# Autodesk Inventor assembly: HoderCutter
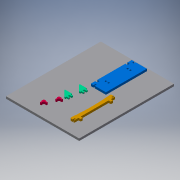
[picture p0: Inventor's stored thumbnail of the model, 180x180]
Saved by Autodesk Inventor 2019 (Build 230136000, 136)
## iProperties
Created: 2018-12-05
Part Number: HoderCutter
Document SubType Name: Assembly
Designer: Administrator
Author: Administrator
## Documents named in this file (6)
- H:\Space\Monster Holder\HoderCutter.iam
- H:\Space\Monster Holder\CuttingBoardPrint.ipt
- H:\Space\Monster Holder\MonsterHolderBase.ipt
- H:\Space\Monster Holder\MonsterHolderSupport1.ipt
- H:\Space\Monster Holder\MonsterHolderSupport2.ipt
- H:\Space\Monster Holder\MonsterHolderSupport3.ipt
## Components (7 placed, 5 different names)
1. CuttingBoardPrint:1 — Mate:1, Mate:2, Mate:3, Mate:4, Mate:5, Mate:6
2. MonsterHolderBase:1 — Mate:1
3. MonsterHolderSupport1:1 — Mate:6
4. MonsterHolderSupport1:2 — Mate:5
5. MonsterHolderSupport2:1 — Mate:2
6. MonsterHolderSupport3:1 — Mate:4
7. MonsterHolderSupport3:2 — Mate:3
## Relationships (6: Mate 6)
- Mate:1: CuttingBoardPrint:1 ↔ MonsterHolderBase:1
- Mate:2: CuttingBoardPrint:1 ↔ MonsterHolderSupport2:1
- Mate:3: CuttingBoardPrint:1 ↔ MonsterHolderSupport3:2
- Mate:4: CuttingBoardPrint:1 ↔ MonsterHolderSupport3:1
- Mate:5: CuttingBoardPrint:1 ↔ MonsterHolderSupport1:2
- Mate:6: CuttingBoardPrint:1 ↔ MonsterHolderSupport1:1
